# Autodesk Inventor assembly: Assembly1
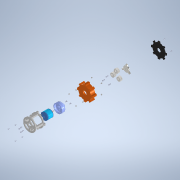
[picture p0: Inventor's stored thumbnail of the model, 180x180]
Saved by Autodesk Inventor 2022 (Build 260153000, 153)
## iProperties
Created: 2022-04-22
Part Number: Assembly1
Document SubType Name: Assembly
Designer: Mlees
Author: Mlees
## Documents named in this file (12)
- C:\Users\Mlees\Desktop\504Engineering\Project_0000\Designs\Design_2\Exported\PRESENTATION\Assembly1.iam
- C:\Users\Mlees\Desktop\504Engineering\Project_0000\Designs\Design_2\Downloads\m100-motor-1.snapshot.1\M100-MOTOR-R1.ipt
- C:\Users\Mlees\Desktop\504Engineering\Project_0000\Designs\Design_2\Created_Parts\Gear_Box_Motor_Support_Bracket.ipt
- C:\Users\Mlees\Desktop\504Engineering\Project_0000\Designs\Design_2\Downloads\91420A116_Steel Phillips Flat Head Screws_M3x6mm.ipt
- C:\Users\Mlees\Desktop\504Engineering\Project_0000\Designs\Design_2\Created_Parts\Gear_Box_Motor_Input.ipt
- C:\Users\Mlees\Desktop\504Engineering\Project_0000\Designs\Design_2\Created_Parts\Gear_Box_Chasis_Lvl_1.ipt
- C:\Users\Mlees\Desktop\504Engineering\Project_0000\Designs\Design_2\Downloads\94180A321_Tapered Heat-Set Inserts for Plastic_M2-5x3.4mm_0-152inmaxhomesize.ipt
- C:\Users\Mlees\Desktop\504Engineering\Project_0000\Designs\Design_2\Downloads\91420A014_Steel Phillips Flat Head Screws_M2-5x5mm.ipt
- C:\Users\Mlees\Desktop\504Engineering\Project_0000\Designs\Design_2\Created_Parts\Gear_Folder\5to1GearCreation_Trial_1\Design Accelerator\Spur Gear23.ipt
- C:\Users\Mlees\Desktop\504Engineering\Project_0000\Designs\Design_2\Created_Parts\Planet_Gear_Output.ipt
- C:\Users\Mlees\Desktop\504Engineering\Project_0000\Designs\Design_2\Downloads\91420A120_Steel Phillips Flat Head ScrewsM3x10mm.ipt
- C:\Users\Mlees\Desktop\504Engineering\Project_0000\Designs\Design_2\Created_Parts\Gear_Box_Chasis_Divider.ipt
## Components (34 placed, 10 different names)
1. M100-MOTOR-R1:1 — Mate:1, Mate:6, Mate:9
2. Gear_Box_Motor_Support_Bracket:1 — Mate:1, Mate:2, Mate:3, Mate:4, Mate:5, Mate:11, Mate:20, Mate:21, Mate:22, Mate:23
3. 91420A116_Steel Phillips Flat Head Screws_M3x6mm:1 — Mate:2
4. 91420A116_Steel Phillips Flat Head Screws_M3x6mm:2 — Mate:3
5. 91420A116_Steel Phillips Flat Head Screws_M3x6mm:3 — Mate:4
6. 91420A116_Steel Phillips Flat Head Screws_M3x6mm:4 — Mate:5
7. Spur Gear1:1 — Mate:6, Mate:7, Mate:8, Mate:9, Mate:10
8. 91420A116_Steel Phillips Flat Head Screws_M3x6mm:5 — Mate:7
9. 91420A116_Steel Phillips Flat Head Screws_M3x6mm:6 — Mate:8
10. Spur Gear2:1 — Mate:10, Mate:11, Mate:12, Mate:13, Mate:14, Mate:15, Mate:16, Mate:17, Mate:18, Mate:19, Mate:24, Mate:25, Mate:26, Mate:34, Mate:35
11. 94180A321_Tapered Heat-Set Inserts for Plastic_M2-5x3.4mm_0-152inmaxhomesize:1 — Mate:12, Flush:3
12. 94180A321_Tapered Heat-Set Inserts for Plastic_M2-5x3.4mm_0-152inmaxhomesize:2 — Mate:13, Flush:2, Flush:3
13. 94180A321_Tapered Heat-Set Inserts for Plastic_M2-5x3.4mm_0-152inmaxhomesize:3 — Mate:14, Flush:1, Flush:2
14. 94180A321_Tapered Heat-Set Inserts for Plastic_M2-5x3.4mm_0-152inmaxhomesize:4 — Mate:15, Flush:1
15. 94180A321_Tapered Heat-Set Inserts for Plastic_M2-5x3.4mm_0-152inmaxhomesize:5 — Mate:19, Flush:4, Flush:6
16. 94180A321_Tapered Heat-Set Inserts for Plastic_M2-5x3.4mm_0-152inmaxhomesize:6 — Mate:18, Flush:6
17. 94180A321_Tapered Heat-Set Inserts for Plastic_M2-5x3.4mm_0-152inmaxhomesize:7 — Mate:17, Flush:4, Flush:5
18. 94180A321_Tapered Heat-Set Inserts for Plastic_M2-5x3.4mm_0-152inmaxhomesize:8 — Mate:16, Flush:5
19. 91420A014_Steel Phillips Flat Head Screws_M2-5x5mm:1 — Mate:21, Flush:7, Flush:9
20. 91420A014_Steel Phillips Flat Head Screws_M2-5x5mm:2 — Mate:22, Flush:8, Flush:9
21. 91420A014_Steel Phillips Flat Head Screws_M2-5x5mm:3 — Mate:23, Flush:8
22. 91420A014_Steel Phillips Flat Head Screws_M2-5x5mm:4 — Mate:20, Flush:7
23. Spur Gear2:2 — Mate:25, Flush:10, Flush:11, Mate:28, Mate:32
24. Spur Gear2:3 — Mate:24, Flush:11, Mate:29, Mate:31
25. Spur Gear2:4 — Mate:26, Flush:10, Mate:27, Mate:30
26. Planet_Gear_Output:1 — Mate:27, Mate:28, Mate:29, Mate:33
27. 91420A120_Steel Phillips Flat Head ScrewsM3x10mm:1 — Mate:30, Flush:12, Flush:13
28. 91420A120_Steel Phillips Flat Head ScrewsM3x10mm:2 — Mate:31, Flush:12
29. 91420A120_Steel Phillips Flat Head ScrewsM3x10mm:3 — Mate:32, Flush:13
30. Gear_Box_Chasis_Divider:1 — Mate:33, Mate:34, Mate:35, Mate:36, Mate:37, Mate:38, Mate:39
31. 91420A014_Steel Phillips Flat Head Screws_M2-5x5mm:5 — Mate:37, Flush:15
32. 91420A014_Steel Phillips Flat Head Screws_M2-5x5mm:6 — Mate:39, Flush:15, Flush:16
33. 91420A014_Steel Phillips Flat Head Screws_M2-5x5mm:7 — Mate:38, Flush:14
34. 91420A014_Steel Phillips Flat Head Screws_M2-5x5mm:8 — Mate:36, Flush:14, Flush:16
## Relationships (55: Mate 39, Flush 16)
- Mate:1: M100-MOTOR-R1:1 ↔ Gear_Box_Motor_Support_Bracket:1
- Mate:2: Gear_Box_Motor_Support_Bracket:1 ↔ 91420A116_Steel Phillips Flat Head Screws_M3x6mm:1
- Mate:3: Gear_Box_Motor_Support_Bracket:1 ↔ 91420A116_Steel Phillips Flat Head Screws_M3x6mm:2
- Mate:4: Gear_Box_Motor_Support_Bracket:1 ↔ 91420A116_Steel Phillips Flat Head Screws_M3x6mm:3
- Mate:5: Gear_Box_Motor_Support_Bracket:1 ↔ 91420A116_Steel Phillips Flat Head Screws_M3x6mm:4
- Mate:6: M100-MOTOR-R1:1 ↔ Spur Gear1:1
- Mate:7: Spur Gear1:1 ↔ 91420A116_Steel Phillips Flat Head Screws_M3x6mm:5
- Mate:8: Spur Gear1:1 ↔ 91420A116_Steel Phillips Flat Head Screws_M3x6mm:6
- Mate:9: M100-MOTOR-R1:1 ↔ Spur Gear1:1
- Mate:10: Spur Gear1:1 ↔ Spur Gear2:1
- Mate:11: Gear_Box_Motor_Support_Bracket:1 ↔ Spur Gear2:1
- Mate:12: Spur Gear2:1 ↔ 94180A321_Tapered Heat-Set Inserts for Plastic_M2-5x3.4mm_0-152inmaxhomesize:1
- Mate:13: Spur Gear2:1 ↔ 94180A321_Tapered Heat-Set Inserts for Plastic_M2-5x3.4mm_0-152inmaxhomesize:2
- Mate:14: Spur Gear2:1 ↔ 94180A321_Tapered Heat-Set Inserts for Plastic_M2-5x3.4mm_0-152inmaxhomesize:3
- Mate:15: Spur Gear2:1 ↔ 94180A321_Tapered Heat-Set Inserts for Plastic_M2-5x3.4mm_0-152inmaxhomesize:4
- Flush:1: 94180A321_Tapered Heat-Set Inserts for Plastic_M2-5x3.4mm_0-152inmaxhomesize:3 ↔ 94180A321_Tapered Heat-Set Inserts for Plastic_M2-5x3.4mm_0-152inmaxhomesize:4
- Flush:2: 94180A321_Tapered Heat-Set Inserts for Plastic_M2-5x3.4mm_0-152inmaxhomesize:2 ↔ 94180A321_Tapered Heat-Set Inserts for Plastic_M2-5x3.4mm_0-152inmaxhomesize:3
- Flush:3: 94180A321_Tapered Heat-Set Inserts for Plastic_M2-5x3.4mm_0-152inmaxhomesize:1 ↔ 94180A321_Tapered Heat-Set Inserts for Plastic_M2-5x3.4mm_0-152inmaxhomesize:2
- Mate:16: Spur Gear2:1 ↔ 94180A321_Tapered Heat-Set Inserts for Plastic_M2-5x3.4mm_0-152inmaxhomesize:8
- Mate:17: Spur Gear2:1 ↔ 94180A321_Tapered Heat-Set Inserts for Plastic_M2-5x3.4mm_0-152inmaxhomesize:7
- Mate:18: Spur Gear2:1 ↔ 94180A321_Tapered Heat-Set Inserts for Plastic_M2-5x3.4mm_0-152inmaxhomesize:6
- Mate:19: Spur Gear2:1 ↔ 94180A321_Tapered Heat-Set Inserts for Plastic_M2-5x3.4mm_0-152inmaxhomesize:5
- Flush:4: 94180A321_Tapered Heat-Set Inserts for Plastic_M2-5x3.4mm_0-152inmaxhomesize:5 ↔ 94180A321_Tapered Heat-Set Inserts for Plastic_M2-5x3.4mm_0-152inmaxhomesize:7
- Flush:5: 94180A321_Tapered Heat-Set Inserts for Plastic_M2-5x3.4mm_0-152inmaxhomesize:7 ↔ 94180A321_Tapered Heat-Set Inserts for Plastic_M2-5x3.4mm_0-152inmaxhomesize:8
- Flush:6: 94180A321_Tapered Heat-Set Inserts for Plastic_M2-5x3.4mm_0-152inmaxhomesize:5 ↔ 94180A321_Tapered Heat-Set Inserts for Plastic_M2-5x3.4mm_0-152inmaxhomesize:6
- Mate:20: Gear_Box_Motor_Support_Bracket:1 ↔ 91420A014_Steel Phillips Flat Head Screws_M2-5x5mm:4
- Mate:21: Gear_Box_Motor_Support_Bracket:1 ↔ 91420A014_Steel Phillips Flat Head Screws_M2-5x5mm:1
- Mate:22: Gear_Box_Motor_Support_Bracket:1 ↔ 91420A014_Steel Phillips Flat Head Screws_M2-5x5mm:2
- Mate:23: Gear_Box_Motor_Support_Bracket:1 ↔ 91420A014_Steel Phillips Flat Head Screws_M2-5x5mm:3
- Flush:7: 91420A014_Steel Phillips Flat Head Screws_M2-5x5mm:1 ↔ 91420A014_Steel Phillips Flat Head Screws_M2-5x5mm:4
- Flush:8: 91420A014_Steel Phillips Flat Head Screws_M2-5x5mm:2 ↔ 91420A014_Steel Phillips Flat Head Screws_M2-5x5mm:3
- Flush:9: 91420A014_Steel Phillips Flat Head Screws_M2-5x5mm:1 ↔ 91420A014_Steel Phillips Flat Head Screws_M2-5x5mm:2
- Mate:24 (16.272 mm): Spur Gear2:1 ↔ Spur Gear2:3
- Mate:25 (16.272 mm): Spur Gear2:1 ↔ Spur Gear2:2
- Mate:26 (16.272 mm): Spur Gear2:1 ↔ Spur Gear2:4
- Flush:10: Spur Gear2:2 ↔ Spur Gear2:4
- Flush:11: Spur Gear2:2 ↔ Spur Gear2:3
- Mate:27: Spur Gear2:4 ↔ Planet_Gear_Output:1
- Mate:28: Spur Gear2:2 ↔ Planet_Gear_Output:1
- Mate:29: Spur Gear2:3 ↔ Planet_Gear_Output:1
- Mate:30: Spur Gear2:4 ↔ 91420A120_Steel Phillips Flat Head ScrewsM3x10mm:1
- Mate:31: Spur Gear2:3 ↔ 91420A120_Steel Phillips Flat Head ScrewsM3x10mm:2
- Mate:32: Spur Gear2:2 ↔ 91420A120_Steel Phillips Flat Head ScrewsM3x10mm:3
- Flush:12: 91420A120_Steel Phillips Flat Head ScrewsM3x10mm:1 ↔ 91420A120_Steel Phillips Flat Head ScrewsM3x10mm:2
- Flush:13: 91420A120_Steel Phillips Flat Head ScrewsM3x10mm:1 ↔ 91420A120_Steel Phillips Flat Head ScrewsM3x10mm:3
- Mate:33: Planet_Gear_Output:1 ↔ Gear_Box_Chasis_Divider:1
- Mate:34: Spur Gear2:1 ↔ Gear_Box_Chasis_Divider:1
- Mate:35: Spur Gear2:1 ↔ Gear_Box_Chasis_Divider:1
- Mate:36: Gear_Box_Chasis_Divider:1 ↔ 91420A014_Steel Phillips Flat Head Screws_M2-5x5mm:8
- Mate:37: Gear_Box_Chasis_Divider:1 ↔ 91420A014_Steel Phillips Flat Head Screws_M2-5x5mm:5
- Mate:38: Gear_Box_Chasis_Divider:1 ↔ 91420A014_Steel Phillips Flat Head Screws_M2-5x5mm:7
- Mate:39: Gear_Box_Chasis_Divider:1 ↔ 91420A014_Steel Phillips Flat Head Screws_M2-5x5mm:6
- Flush:14: 91420A014_Steel Phillips Flat Head Screws_M2-5x5mm:7 ↔ 91420A014_Steel Phillips Flat Head Screws_M2-5x5mm:8
- Flush:15: 91420A014_Steel Phillips Flat Head Screws_M2-5x5mm:5 ↔ 91420A014_Steel Phillips Flat Head Screws_M2-5x5mm:6
- Flush:16: 91420A014_Steel Phillips Flat Head Screws_M2-5x5mm:6 ↔ 91420A014_Steel Phillips Flat Head Screws_M2-5x5mm:8
